# Autodesk Inventor assembly: New redesign Assembly
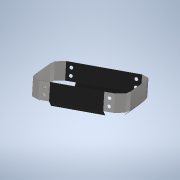
[picture p0: Inventor's stored thumbnail of the model, 180x180]
Saved by Autodesk Inventor 2020 (Build 240168000, 168)
## iProperties
Created: 2022-07-17
Part Number: New redesign Assembly
Document SubType Name: Assembly
Designer: karimi2
Author: karimi2
## Documents named in this file (3)
- C:\Users\karimi2\Documents\PROJECT\src\New redesign Assembly.iam
- C:\Users\karimi2\Documents\PROJECT\src\New front.ipt
- C:\Users\karimi2\Documents\PROJECT\src\New side.ipt
## Components (4 placed, 2 different names)
1. New front:1 — Mate:1, Mate:2, Mate:3, Mate:7, Mate:8, Mate:9
2. New side:1 — Mate:1, Mate:2, Mate:3, Mate:4, Mate:5, Mate:6
3. New front:2 — Mate:4, Mate:5, Mate:6
4. New side:2 — Mate:7, Mate:8, Mate:9
## Relationships (9: Mate 9)
- Mate:1: New front:1 ↔ New side:1
- Mate:2: New front:1 ↔ New side:1
- Mate:3: New front:1 ↔ New side:1
- Mate:4: New side:1 ↔ New front:2
- Mate:5: New side:1 ↔ New front:2
- Mate:6: New side:1 ↔ New front:2
- Mate:7: New front:1 ↔ New side:2
- Mate:8: New front:1 ↔ New side:2
- Mate:9: New front:1 ↔ New side:2
